# Autodesk Inventor assembly: Esmeril Assy
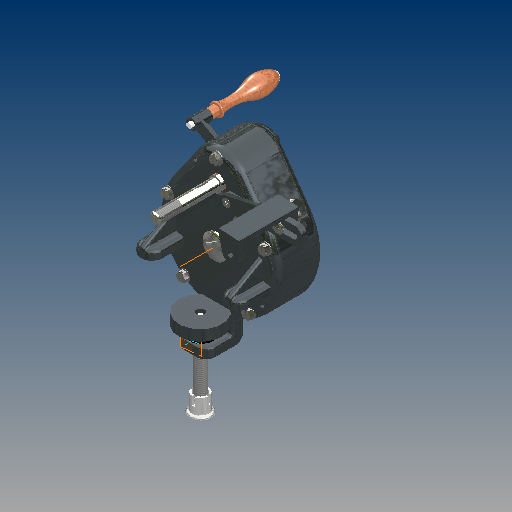
[picture p0: Inventor's stored thumbnail of the model, 512x512]
Saved by Autodesk Inventor 2020 (Build 240168000, 168)
## iProperties
Created: 2019-11-22
Part Number: Esmeril Assy
Document SubType Name: Assembly
Designer: gerar
Author: gerar
## Documents named in this file (16)
- C:\Users\gerar\OneDrive - Instituto Tecnologico y de Estudios Superiores de Monterrey\TEC\Semestre XI\Dibujo Computarizado\Archivos de Inventor\Esmeril\Esmeril Assy.iam
- C:\Users\gerar\OneDrive - Instituto Tecnologico y de Estudios Superiores de Monterrey\TEC\Semestre XI\Dibujo Computarizado\Archivos de Inventor\Esmeril\Cubierta.ipt
- C:\Users\gerar\OneDrive - Instituto Tecnologico y de Estudios Superiores de Monterrey\TEC\Semestre XI\Dibujo Computarizado\Archivos de Inventor\Esmeril\Buje de la Flecha.ipt
- C:\Users\gerar\OneDrive - Instituto Tecnologico y de Estudios Superiores de Monterrey\TEC\Semestre XI\Dibujo Computarizado\Archivos de Inventor\Esmeril\Flecha del engrane.ipt
- C:\Users\gerar\OneDrive - Instituto Tecnologico y de Estudios Superiores de Monterrey\TEC\Semestre XI\Dibujo Computarizado\Archivos de Inventor\Esmeril\Pinion.ipt
- C:\Users\gerar\OneDrive - Instituto Tecnologico y de Estudios Superiores de Monterrey\TEC\Semestre XI\Dibujo Computarizado\Archivos de Inventor\Esmeril\Spur Gear11.ipt
- C:\Users\gerar\OneDrive - Instituto Tecnologico y de Estudios Superiores de Monterrey\TEC\Semestre XI\Dibujo Computarizado\Archivos de Inventor\Esmeril\Caja1.ipt
- C:\Users\gerar\OneDrive - Instituto Tecnologico y de Estudios Superiores de Monterrey\TEC\Semestre XI\Dibujo Computarizado\Archivos de Inventor\Esmeril\Manivela.ipt
- C:\Users\gerar\OneDrive - Instituto Tecnologico y de Estudios Superiores de Monterrey\TEC\Semestre XI\Dibujo Computarizado\Archivos de Inventor\Esmeril\Mango.ipt
- C:\Users\gerar\OneDrive - Instituto Tecnologico y de Estudios Superiores de Monterrey\TEC\Semestre XI\Dibujo Computarizado\Archivos de Inventor\Esmeril\Pasador del Mango.ipt
- C:\Users\gerar\OneDrive\Documentos\Inventor\Content Center Files\R2020\es-ES\ANSI B18.6.3(49)\ANSI B18.6.3 - 1_4 - 20 x 1 1_2(5).ipt
- C:\Users\gerar\OneDrive - Instituto Tecnologico y de Estudios Superiores de Monterrey\TEC\Semestre XI\Dibujo Computarizado\Archivos de Inventor\Esmeril\Tornillo de apriete.ipt
- C:\Users\gerar\OneDrive - Instituto Tecnologico y de Estudios Superiores de Monterrey\TEC\Semestre XI\Dibujo Computarizado\Archivos de Inventor\Esmeril\Disco de Apriete.ipt
- C:\Users\gerar\OneDrive - Instituto Tecnologico y de Estudios Superiores de Monterrey\TEC\Semestre XI\Dibujo Computarizado\Archivos de Inventor\Esmeril\Clamp Knob.ipt
- C:\Users\gerar\OneDrive - Instituto Tecnologico y de Estudios Superiores de Monterrey\TEC\Semestre XI\Dibujo Computarizado\Archivos de Inventor\Esmeril\ARM\ARM.iam
- C:\Users\gerar\OneDrive\Documentos\Inventor\Content Center Files\R2020\es-ES\ANSI B18.6.3(01)\ANSI B18.6.3 - 10-24 UNC - 0.5625(33).ipt
## Components (23 placed, 15 different names)
1. Cubierta:1 — Coincidencia:1, Coincidencia:2, Insertar:1, Coincidencia:9, Insertar:5, Insertar:6, Insertar:7, Insertar:8, Insertar:9, Coincidencia:14, Coincidencia:18, Coincidencia:19, Coincidencia:20
2. Buje de la Flecha:1 — Coincidencia:2, Coincidencia:3
3. Buje de la Flecha:2 — Coincidencia:1, Coincidencia:5
4. Flecha del engrane:1 — Insertar:1, Coincidencia:4, Nivelación:1, Coincidencia:8, Insertar:4, Nivelación:2
5. Shaft:1 — Coincidencia:3, 48/12, Coincidencia:7
6. Spur Gear1:1 — Coincidencia:4, Coincidencia:5, Nivelación:1, 48/12
7. Caja1:1 — Coincidencia:6, Insertar:2, Insertar:3, Coincidencia:9
8. Buje de la Flecha:3 — Coincidencia:6, Insertar:3, Coincidencia:7
9. Buje de la Flecha:4 — Insertar:2, Coincidencia:8
10. Manivela:1 — Insertar:4, Nivelación:2, Coincidencia:10, Coincidencia:11
11. Mango:1 — Coincidencia:10, Coincidencia:11, Coincidencia:12, Coincidencia:13
12. Pasador del Mango:1 — Coincidencia:12, Coincidencia:13
13. Tornillo para maquinaria para arandela de cabeza hex. ranurada - Pulgadas 1/4 - 20 x 1 1/2:1 — Insertar:5
14. Tornillo para maquinaria para arandela de cabeza hex. ranurada - Pulgadas 1/4 - 20 x 1 1/2:2 — Insertar:6
15. Tornillo para maquinaria para arandela de cabeza hex. ranurada - Pulgadas 1/4 - 20 x 1 1/2:3 — Insertar:7
16. Tornillo para maquinaria para arandela de cabeza hex. ranurada - Pulgadas 1/4 - 20 x 1 1/2:4 — Insertar:8
17. Tornillo para maquinaria para arandela de cabeza hex. ranurada - Pulgadas 1/4 - 20 x 1 1/2:5 — Insertar:9
18. Tornillo de apriete:1 — Coincidencia:14, Coincidencia:15, Tangente:1, Coincidencia:16, Coincidencia:17
19. Disco de Apriete:1 — Coincidencia:15, Tangente:1
20. Clamp Knob:1 — Coincidencia:16, Coincidencia:17
21. ARM:1 [sub-assembly] — Coincidencia:18, Coincidencia:19, Coincidencia:20, Coincidencia:21, Coincidencia:22, Nivelación:3, Nivelación:4
22. Tornillo para maquinaria de cabeza plana avellanada con hueco cruciforme a 100° - Tipo IA - Pulgadas 10-24 UNC x 0.5625:1 — Coincidencia:21, Nivelación:3
23. Tornillo para maquinaria de cabeza plana avellanada con hueco cruciforme a 100° - Tipo IA - Pulgadas 10-24 UNC x 0.5625:2 — Coincidencia:22, Nivelación:4
## Relationships (37: Mate 22, Insert 9, Flush 4, RelateRotation 1, Tangent 1)
- Coincidencia:1 [Mate]: Cubierta:1 ↔ Buje de la Flecha:2
- Coincidencia:2 [Mate]: Cubierta:1 ↔ Buje de la Flecha:1
- Insertar:1: Cubierta:1 ↔ Flecha del engrane:1
- Coincidencia:3 [Mate]: Buje de la Flecha:1 ↔ Shaft:1
- Coincidencia:4 [Mate]: Flecha del engrane:1 ↔ Spur Gear1:1
- Coincidencia:5 [Mate]: Buje de la Flecha:2 ↔ Spur Gear1:1
- Nivelación:1 [Flush]: Flecha del engrane:1 ↔ Spur Gear1:1
- 48/12 [RelateRotation] (1 ul): Shaft:1 ↔ Spur Gear1:1
- Coincidencia:6 [Mate]: Caja1:1 ↔ Buje de la Flecha:3
- Insertar:2: Caja1:1 ↔ Buje de la Flecha:4
- Insertar:3: Caja1:1 ↔ Buje de la Flecha:3
- Coincidencia:7 [Mate]: Shaft:1 ↔ Buje de la Flecha:3
- Coincidencia:8 [Mate]: Flecha del engrane:1 ↔ Buje de la Flecha:4
- Coincidencia:9 [Mate]: Cubierta:1 ↔ Caja1:1
- Insertar:4: Flecha del engrane:1 ↔ Manivela:1
- Nivelación:2 [Flush]: Flecha del engrane:1 ↔ Manivela:1
- Coincidencia:10 [Mate]: Manivela:1 ↔ Mango:1
- Coincidencia:11 [Mate]: Manivela:1 ↔ Mango:1
- Coincidencia:12 [Mate]: Mango:1 ↔ Pasador del Mango:1
- Coincidencia:13 [Mate]: Mango:1 ↔ Pasador del Mango:1
- Insertar:5: Cubierta:1 ↔ Tornillo para maquinaria para arandela de cabeza hex. ranurada - Pulgadas 1/4 - 20 x 1 1/2:1
- Insertar:6: Cubierta:1 ↔ Tornillo para maquinaria para arandela de cabeza hex. ranurada - Pulgadas 1/4 - 20 x 1 1/2:2
- Insertar:7: Cubierta:1 ↔ Tornillo para maquinaria para arandela de cabeza hex. ranurada - Pulgadas 1/4 - 20 x 1 1/2:3
- Insertar:8: Cubierta:1 ↔ Tornillo para maquinaria para arandela de cabeza hex. ranurada - Pulgadas 1/4 - 20 x 1 1/2:4
- Insertar:9: Cubierta:1 ↔ Tornillo para maquinaria para arandela de cabeza hex. ranurada - Pulgadas 1/4 - 20 x 1 1/2:5
- Coincidencia:14 [Mate]: Cubierta:1 ↔ Tornillo de apriete:1
- Coincidencia:15 [Mate]: Tornillo de apriete:1 ↔ Disco de Apriete:1
- Tangente:1: Tornillo de apriete:1 ↔ Disco de Apriete:1
- Coincidencia:16 [Mate]: Tornillo de apriete:1 ↔ Clamp Knob:1
- Coincidencia:17 [Mate]: Tornillo de apriete:1 ↔ Clamp Knob:1
- Coincidencia:18 [Mate]: Cubierta:1 ↔ ARM:1
- Coincidencia:19 [Mate]: Cubierta:1 ↔ ARM:1
- Coincidencia:20 [Mate]: Cubierta:1 ↔ ARM:1
- Coincidencia:21 [Mate]: ARM:1 ↔ Tornillo para maquinaria de cabeza plana avellanada con hueco cruciforme a 100° - Tipo IA - Pulgadas 10-24 UNC x 0.5625:1
- Coincidencia:22 [Mate]: ARM:1 ↔ Tornillo para maquinaria de cabeza plana avellanada con hueco cruciforme a 100° - Tipo IA - Pulgadas 10-24 UNC x 0.5625:2
- Nivelación:3 [Flush]: ARM:1 ↔ Tornillo para maquinaria de cabeza plana avellanada con hueco cruciforme a 100° - Tipo IA - Pulgadas 10-24 UNC x 0.5625:1
- Nivelación:4 [Flush]: ARM:1 ↔ Tornillo para maquinaria de cabeza plana avellanada con hueco cruciforme a 100° - Tipo IA - Pulgadas 10-24 UNC x 0.5625:2
